# Autodesk Inventor assembly: In-Robot Assembly Full
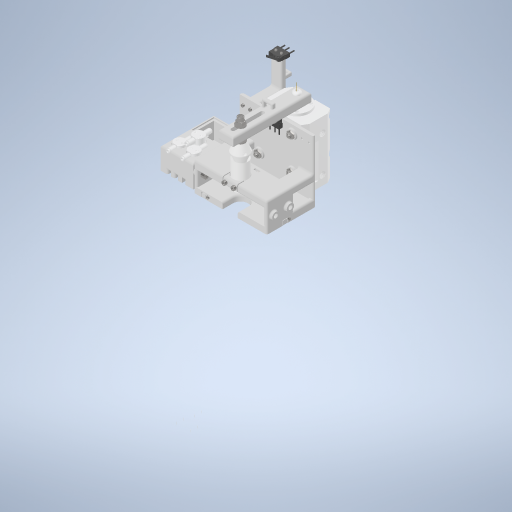
[picture p0: Inventor's stored thumbnail of the model, 512x512]
Saved by Autodesk Inventor 2024.1 (Build 281209000, 209)
## iProperties
Created: 2025-03-13
Part Number: In-Robot Assembly Full
Document SubType Name: Assembly
Designer: pab2
Author: pab2
## Documents named in this file (29)
- C:\Users\pab2\Documents\GitHub\AFL-hardware-devel\CAD-NewOrgScheme\AFL-101-(LoaderV2)\In-Robot Assembly Full.iam
- C:\Users\pab2\Documents\GitHub\AFL-hardware-devel\CAD-NewOrgScheme\AFL-101-(LoaderV2)\002-(CatchCarrierAssy)\AFL-101-002-01-0E CatchlessCatchHolder-Braced-For1inCatch-Sidebar-Lowered.ipt
- C:\Users\pab2\Documents\GitHub\AFL-hardware-devel\CAD-NewOrgScheme\AFL-101-(LoaderV2)\002-(CatchCarrierAssy)\AFL-101-002-01-4E RetainerNut.ipt
- C:\Users\pab2\Documents\GitHub\AFL-hardware-devel\CAD-NewOrgScheme\AFL-101-(LoaderV2)\002-(CatchCarrierAssy)\AFL-101-002-01-1A full-up microswitch arm.ipt
- C:\Users\pab2\Documents\GitHub\AFL-hardware-devel\CAD-NewOrgScheme\AFL-101-(LoaderV2)\002-(CatchCarrierAssy)\AFL-101-002-01-2B Elevator arm r2.ipt
- C:\Users\pab2\Documents\GitHub\AFL-hardware-devel\CAD-NewOrgScheme\AFL-101-(LoaderV2)\002-(CatchCarrierAssy)\AFL-101-002-01-3B CatchHolderNut.ipt
- C:\Users\pab2\Documents\GitHub\AFL-hardware-devel\CAD-NewOrgScheme\AFL-101-(LoaderV2)\001-(CatchAssy)\AFL-101-001-02-0C catch vertical seal-tighttol-thread - SANS.ipt
- C:\Users\pab2\Documents\GitHub\AFL-hardware-devel\CAD-NewOrgScheme\AFL-101-(LoaderV2)\001-(CatchAssy)\AFL-101-001-02-1C piston badflowchannel-1-16in-thread - neutron - 65flowchan.ipt
- C:\Users\pab2\Documents\GitHub\AFL-hardware-devel\CAD-NewOrgScheme\AFL-101-(LoaderV2)\003-(ValveBox)\AFL-101-003-01-0C Valve Holder-3valve-withwirebox-fortappedholes.ipt
- C:\Users\pab2\Downloads\50185A34_Air-Powered Hold-Down Fixture Clamp\50185A34_Air-Powered Hold-Down Fixture Clamp.ipt
- C:\Users\pab2\Downloads\5001T38_Miniature Solenoid On-Off Valve\5001T38_Miniature Solenoid On-Off Valve.ipt
- C:\Users\pab2\Downloads\8085T18_Subminiature Wet-Location Snap-Acting Switch\8085T18_Subminiature Wet-Location Snap-Acting Switch.ipt
- C:\Users\pab2\Documents\Inventor\Content Center Files\R2024\en-US\ANSI B18.2.2(09)\ANSI B18.2.2 - 1_4 - 20(2).ipt
- C:\Users\pab2\Documents\Inventor\Content Center Files\R2024\en-US\ANSI B18.3(05)\ANSI B18.3 - 1_4-20 UNC - 1.75(31).ipt
- C:\Users\pab2\Documents\Inventor\Content Center Files\R2024\en-US\ANSI B18.3(05)\ANSI B18.3 - 1_4-20 UNC - 0.25(31).ipt
- C:\Users\pab2\Documents\Inventor\Content Center Files\R2024\en-US\ANSI B18.3(05)\ANSI B18.3 - 8-32 UNC - 1.75(31).ipt
- C:\Users\pab2\Documents\Inventor\Content Center Files\R2024\en-US\ANSI B18.2.2(06)\ANSI B18.2.2 - 8 - 32(06).ipt
- C:\Users\pab2\Documents\Inventor\Content Center Files\R2024\en-US\ANSI B18.3(05)\ANSI B18.3 - 4-40 UNC - 0.25(31).ipt
- C:\Users\pab2\Documents\Inventor\Content Center Files\R2024\en-US\ANSI B18.3(05)\ANSI B18.3 - 2-56 UNC - 0.15625(31).ipt
- C:\Users\pab2\Documents\Inventor\Content Center Files\R2024\en-US\ANSI B18.3(05)\ANSI B18.3 - 4-40 UNC - 0.5(31).ipt
- C:\Users\pab2\Downloads\5779K241_Push-to-Connect Tube Fitting for Air\5779K241_Push-to-Connect Tube Fitting for Air.ipt
- C:\Users\pab2\Documents\Inventor\Content Center Files\R2024\en-US\ASTM F436(1)\ASTM F436 - 1_4(1).ipt
- C:\Users\pab2\Documents\Inventor\Content Center Files\R2024\en-US\ANSI B18.3(05)\ANSI B18.3 - 1_4-20 UNC - 1.5(31).ipt
- C:\Users\pab2\Documents\GitHub\AFL-hardware-devel\CAD-NewOrgScheme\AFL-101-(LoaderV2)\In-Robot Assembly Full\AIP\FEA\f06gvksv4.fins
- C:\Users\pab2\Documents\GitHub\AFL-hardware-devel\CAD-NewOrgScheme\AFL-101-(LoaderV2)\In-Robot Assembly Full\AIP\FEA\f06gvksw0.fsat
- C:\Users\pab2\Documents\GitHub\AFL-hardware-devel\CAD-NewOrgScheme\AFL-101-(LoaderV2)\In-Robot Assembly Full\AIP\FEA\f06gvksw0.ftes
- C:\Users\pab2\Documents\GitHub\AFL-hardware-devel\CAD-NewOrgScheme\AFL-101-(LoaderV2)\In-Robot Assembly Full\AIP\FEA\f06gvksw0.fwiz
- C:\Users\pab2\Documents\GitHub\AFL-hardware-devel\CAD-NewOrgScheme\AFL-101-(LoaderV2)\In-Robot Assembly Full\AIP\FEA\f06gvkta8.fmsh
- C:\Users\pab2\Documents\GitHub\AFL-hardware-devel\CAD-NewOrgScheme\AFL-101-(LoaderV2)\In-Robot Assembly Full\AIP\FEA\f06gvkta9.fres
## Components (49 placed, 22 different names)
1. AFL-101-002-01-0E CatchlessCatchHolder-Braced-For1inCatch-Sidebar-Lowered:1 — Mate:1, Mate:2, Mate:3, Mate:4, Mate:5, Mate:6, Mate:10, Flush:1, Mate:11, Flush:2, Mate:12, Mate:13, Mate:14, Mate:15, Mate:16, Mate:17, Mate:27, Mate:28, Mate:29, Insert:1, Insert:2, Insert:3, Insert:4, Insert:9, Insert:10, Insert:11, Insert:14, Insert:15, Insert:16, Insert:17, Insert:22, Insert:23
2. AFL-101-002-01-4E RetainerNut:1 — Mate:11, Flush:2
3. AFL-101-002-01-4E RetainerNut:2 — Mate:10, Flush:1
4. AFL-101-002-01-1A full-up microswitch arm:1 — Mate:12, Mate:13, Mate:14, Mate:24, Mate:25, Mate:26
5. AFL-101-002-01-2B Elevator arm r2:1 — Mate:18, Angle:1, Mate:42, Mate:44
6. AFL-101-002-01-3B CatchHolderNut:1 — Mate:7, Mate:8, Mate:9, Insert:12, Insert:13
7. AFL-101-001-02-0C catch vertical seal-tighttol-thread - SANS:1 — Mate:4, Mate:5, Mate:6, Mate:7, Mate:8, Mate:9, Mate:19
8. AFL-101-001-02-1C piston badflowchannel-1-16in-thread - neutron - 65flowchan:1 — Mate:19, Insert:24, Mate:43, Mate:44
9. AFL-101-003-01-0C Valve Holder-3valve-withwirebox-fortappedholes:1 — Mate:1, Mate:2, Mate:3, Mate:21, Mate:22, Mate:23
10. 50185A34_Air-Powered Hold-Down Fixture Clamp:1 — Mate:15, Mate:16, Mate:17, Mate:18, Angle:1, Insert:5, Insert:6, Insert:7, Insert:8
11. 5001T38_Miniature Solenoid On-Off Valve:1 — Mate:22, Mate:34, Mate:35, Mate:40, Mate:41
12. 5001T38_Miniature Solenoid On-Off Valve:2 — Mate:21, Mate:32, Mate:33, Mate:36, Mate:37
13. 5001T38_Miniature Solenoid On-Off Valve:3 — Mate:23, Mate:30, Mate:31, Mate:38, Mate:39
14. 8085T18_Subminiature Wet-Location Snap-Acting Switch:1 — Mate:27, Mate:28, Mate:29, Insert:20, Insert:21
15. 8085T18_Subminiature Wet-Location Snap-Acting Switch:2 — Mate:24, Mate:25, Mate:26, Insert:18, Insert:19
16. Hex Nut - Inch 1/4 - 20:1 — Insert:1
17. Hex Nut - Inch 1/4 - 20:2 — Insert:2
18. Hex Nut - Inch 1/4 - 20:3 — Insert:3
19. Hex Nut - Inch 1/4 - 20:4 — Insert:4
20. Hexagon Socket Head Cap Screw - Inch 1/4 - 20 UNC - 1 3/4:1 — Insert:5
21. Hexagon Socket Head Cap Screw - Inch 1/4 - 20 UNC - 1 3/4:2 — Insert:6
22. Hexagon Socket Head Cap Screw - Inch 1/4 - 20 UNC - 1 3/4:3 — Insert:7
23. Hexagon Socket Head Cap Screw - Inch 1/4 - 20 UNC - 1 3/4:4 — Insert:8
24. Hexagon Socket Head Cap Screw - Inch 1/4 - 20 UNC - 1/4:1 — Insert:9
25. Hexagon Socket Head Cap Screw - Inch 1/4 - 20 UNC - 1/4:2 — Insert:10
26. Hexagon Socket Head Cap Screw - Inch 1/4 - 20 UNC - 1/4:3 — Insert:11
27. Hexagon Socket Head Cap Screw - Inch No. 8 - 32 UNC - 1 3/4:1 — Insert:12
28. Hexagon Socket Head Cap Screw - Inch No. 8 - 32 UNC - 1 3/4:2 — Insert:13
29. Hex Machine Screw Nut - Inch 8 - 32:1 — Insert:14
30. Hex Machine Screw Nut - Inch 8 - 32:2 — Insert:15
31. Hexagon Socket Head Cap Screw - Inch No. 4 - 40 UNC - 1/4:2 — Insert:16
32. Hexagon Socket Head Cap Screw - Inch No. 4 - 40 UNC - 1/4:1 — Insert:17
33. Hexagon Socket Head Cap Screw - Inch No. 2 - 56 UNC - 5/32:1 — Insert:18
34. Hexagon Socket Head Cap Screw - Inch No. 2 - 56 UNC - 5/32:2 — Insert:19
35. Hexagon Socket Head Cap Screw - Inch No. 2 - 56 UNC - 5/32:3 — Insert:20
36. Hexagon Socket Head Cap Screw - Inch No. 2 - 56 UNC - 5/32:4 — Insert:21
37. Hexagon Socket Head Cap Screw - Inch No. 4 - 40 UNC - 1/2:2 — Insert:22
38. Hexagon Socket Head Cap Screw - Inch No. 4 - 40 UNC - 1/2:1 — Insert:23
39. 5779K241_Push-to-Connect Tube Fitting for Air:1 — Mate:32, Mate:33
40. 5779K241_Push-to-Connect Tube Fitting for Air:2 — Mate:36, Mate:37
41. 5779K241_Push-to-Connect Tube Fitting for Air:3 — Mate:34, Mate:35
42. 5779K241_Push-to-Connect Tube Fitting for Air:4 — Mate:30, Mate:31
43. 5779K241_Push-to-Connect Tube Fitting for Air:5 — Mate:38, Mate:39
44. 5779K241_Push-to-Connect Tube Fitting for Air:6 — Mate:40, Mate:41
45. Circular Washer (Inch) 1/4:1 — Insert:24, Insert:25
46. Hex Nut - Inch 1/4 - 20:5 — Insert:25
47. Circular Washer (Inch) 1/4:2 — Mate:42, Mate:43, Insert:26
48. Hex Nut - Inch 1/4 - 20:6 — Insert:26, Insert:27
49. Hexagon Socket Head Cap Screw - Inch 1/4 - 20 UNC - 1 1/2:1 — Insert:27
## Relationships (73: Mate 43, Insert 27, Flush 2, Angle 1)
- Mate:1: AFL-101-002-01-0E CatchlessCatchHolder-Braced-For1inCatch-Sidebar-Lowered:1 ↔ AFL-101-003-01-0C Valve Holder-3valve-withwirebox-fortappedholes:1
- Mate:2: AFL-101-002-01-0E CatchlessCatchHolder-Braced-For1inCatch-Sidebar-Lowered:1 ↔ AFL-101-003-01-0C Valve Holder-3valve-withwirebox-fortappedholes:1
- Mate:3: AFL-101-002-01-0E CatchlessCatchHolder-Braced-For1inCatch-Sidebar-Lowered:1 ↔ AFL-101-003-01-0C Valve Holder-3valve-withwirebox-fortappedholes:1
- Mate:4: AFL-101-002-01-0E CatchlessCatchHolder-Braced-For1inCatch-Sidebar-Lowered:1 ↔ AFL-101-001-02-0C catch vertical seal-tighttol-thread - SANS:1
- Mate:5: AFL-101-002-01-0E CatchlessCatchHolder-Braced-For1inCatch-Sidebar-Lowered:1 ↔ AFL-101-001-02-0C catch vertical seal-tighttol-thread - SANS:1
- Mate:6: AFL-101-002-01-0E CatchlessCatchHolder-Braced-For1inCatch-Sidebar-Lowered:1 ↔ AFL-101-001-02-0C catch vertical seal-tighttol-thread - SANS:1
- Mate:7: AFL-101-002-01-3B CatchHolderNut:1 ↔ AFL-101-001-02-0C catch vertical seal-tighttol-thread - SANS:1
- Mate:8: AFL-101-002-01-3B CatchHolderNut:1 ↔ AFL-101-001-02-0C catch vertical seal-tighttol-thread - SANS:1
- Mate:9: AFL-101-002-01-3B CatchHolderNut:1 ↔ AFL-101-001-02-0C catch vertical seal-tighttol-thread - SANS:1
- Mate:10: AFL-101-002-01-0E CatchlessCatchHolder-Braced-For1inCatch-Sidebar-Lowered:1 ↔ AFL-101-002-01-4E RetainerNut:2
- Flush:1: AFL-101-002-01-0E CatchlessCatchHolder-Braced-For1inCatch-Sidebar-Lowered:1 ↔ AFL-101-002-01-4E RetainerNut:2
- Mate:11: AFL-101-002-01-0E CatchlessCatchHolder-Braced-For1inCatch-Sidebar-Lowered:1 ↔ AFL-101-002-01-4E RetainerNut:1
- Flush:2: AFL-101-002-01-0E CatchlessCatchHolder-Braced-For1inCatch-Sidebar-Lowered:1 ↔ AFL-101-002-01-4E RetainerNut:1
- Mate:12: AFL-101-002-01-0E CatchlessCatchHolder-Braced-For1inCatch-Sidebar-Lowered:1 ↔ AFL-101-002-01-1A full-up microswitch arm:1
- Mate:13: AFL-101-002-01-0E CatchlessCatchHolder-Braced-For1inCatch-Sidebar-Lowered:1 ↔ AFL-101-002-01-1A full-up microswitch arm:1
- Mate:14: AFL-101-002-01-0E CatchlessCatchHolder-Braced-For1inCatch-Sidebar-Lowered:1 ↔ AFL-101-002-01-1A full-up microswitch arm:1
- Mate:15: AFL-101-002-01-0E CatchlessCatchHolder-Braced-For1inCatch-Sidebar-Lowered:1 ↔ 50185A34_Air-Powered Hold-Down Fixture Clamp:1
- Mate:16: AFL-101-002-01-0E CatchlessCatchHolder-Braced-For1inCatch-Sidebar-Lowered:1 ↔ 50185A34_Air-Powered Hold-Down Fixture Clamp:1
- Mate:17: AFL-101-002-01-0E CatchlessCatchHolder-Braced-For1inCatch-Sidebar-Lowered:1 ↔ 50185A34_Air-Powered Hold-Down Fixture Clamp:1
- Mate:18: AFL-101-002-01-2B Elevator arm r2:1 ↔ 50185A34_Air-Powered Hold-Down Fixture Clamp:1
- Angle:1 (90 deg): AFL-101-002-01-2B Elevator arm r2:1 ↔ 50185A34_Air-Powered Hold-Down Fixture Clamp:1
- Mate:19: AFL-101-001-02-0C catch vertical seal-tighttol-thread - SANS:1 ↔ AFL-101-001-02-1C piston badflowchannel-1-16in-thread - neutron - 65flowchan:1
- Mate:21: AFL-101-003-01-0C Valve Holder-3valve-withwirebox-fortappedholes:1 ↔ 5001T38_Miniature Solenoid On-Off Valve:2
- Mate:22: AFL-101-003-01-0C Valve Holder-3valve-withwirebox-fortappedholes:1 ↔ 5001T38_Miniature Solenoid On-Off Valve:1
- Mate:23: AFL-101-003-01-0C Valve Holder-3valve-withwirebox-fortappedholes:1 ↔ 5001T38_Miniature Solenoid On-Off Valve:3
- Mate:24: AFL-101-002-01-1A full-up microswitch arm:1 ↔ 8085T18_Subminiature Wet-Location Snap-Acting Switch:2
- Mate:25: AFL-101-002-01-1A full-up microswitch arm:1 ↔ 8085T18_Subminiature Wet-Location Snap-Acting Switch:2
- Mate:26: AFL-101-002-01-1A full-up microswitch arm:1 ↔ 8085T18_Subminiature Wet-Location Snap-Acting Switch:2
- Mate:27: AFL-101-002-01-0E CatchlessCatchHolder-Braced-For1inCatch-Sidebar-Lowered:1 ↔ 8085T18_Subminiature Wet-Location Snap-Acting Switch:1
- Mate:28: AFL-101-002-01-0E CatchlessCatchHolder-Braced-For1inCatch-Sidebar-Lowered:1 ↔ 8085T18_Subminiature Wet-Location Snap-Acting Switch:1
- Mate:29: AFL-101-002-01-0E CatchlessCatchHolder-Braced-For1inCatch-Sidebar-Lowered:1 ↔ 8085T18_Subminiature Wet-Location Snap-Acting Switch:1
- Insert:1: AFL-101-002-01-0E CatchlessCatchHolder-Braced-For1inCatch-Sidebar-Lowered:1 ↔ Hex Nut - Inch 1/4 - 20:1
- Insert:2: AFL-101-002-01-0E CatchlessCatchHolder-Braced-For1inCatch-Sidebar-Lowered:1 ↔ Hex Nut - Inch 1/4 - 20:2
- Insert:3: AFL-101-002-01-0E CatchlessCatchHolder-Braced-For1inCatch-Sidebar-Lowered:1 ↔ Hex Nut - Inch 1/4 - 20:3
- Insert:4: AFL-101-002-01-0E CatchlessCatchHolder-Braced-For1inCatch-Sidebar-Lowered:1 ↔ Hex Nut - Inch 1/4 - 20:4
- Insert:5: 50185A34_Air-Powered Hold-Down Fixture Clamp:1 ↔ Hexagon Socket Head Cap Screw - Inch 1/4 - 20 UNC - 1 3/4:1
- Insert:6: 50185A34_Air-Powered Hold-Down Fixture Clamp:1 ↔ Hexagon Socket Head Cap Screw - Inch 1/4 - 20 UNC - 1 3/4:2
- Insert:7: 50185A34_Air-Powered Hold-Down Fixture Clamp:1 ↔ Hexagon Socket Head Cap Screw - Inch 1/4 - 20 UNC - 1 3/4:3
- Insert:8: 50185A34_Air-Powered Hold-Down Fixture Clamp:1 ↔ Hexagon Socket Head Cap Screw - Inch 1/4 - 20 UNC - 1 3/4:4
- Insert:9: AFL-101-002-01-0E CatchlessCatchHolder-Braced-For1inCatch-Sidebar-Lowered:1 ↔ Hexagon Socket Head Cap Screw - Inch 1/4 - 20 UNC - 1/4:1
- Insert:10: AFL-101-002-01-0E CatchlessCatchHolder-Braced-For1inCatch-Sidebar-Lowered:1 ↔ Hexagon Socket Head Cap Screw - Inch 1/4 - 20 UNC - 1/4:2
- Insert:11: AFL-101-002-01-0E CatchlessCatchHolder-Braced-For1inCatch-Sidebar-Lowered:1 ↔ Hexagon Socket Head Cap Screw - Inch 1/4 - 20 UNC - 1/4:3
- Insert:12: AFL-101-002-01-3B CatchHolderNut:1 ↔ Hexagon Socket Head Cap Screw - Inch No. 8 - 32 UNC - 1 3/4:1
- Insert:13: AFL-101-002-01-3B CatchHolderNut:1 ↔ Hexagon Socket Head Cap Screw - Inch No. 8 - 32 UNC - 1 3/4:2
- Insert:14: AFL-101-002-01-0E CatchlessCatchHolder-Braced-For1inCatch-Sidebar-Lowered:1 ↔ Hex Machine Screw Nut - Inch 8 - 32:1
- Insert:15: AFL-101-002-01-0E CatchlessCatchHolder-Braced-For1inCatch-Sidebar-Lowered:1 ↔ Hex Machine Screw Nut - Inch 8 - 32:2
- Insert:16: AFL-101-002-01-0E CatchlessCatchHolder-Braced-For1inCatch-Sidebar-Lowered:1 ↔ Hexagon Socket Head Cap Screw - Inch No. 4 - 40 UNC - 1/4:2
- Insert:17: AFL-101-002-01-0E CatchlessCatchHolder-Braced-For1inCatch-Sidebar-Lowered:1 ↔ Hexagon Socket Head Cap Screw - Inch No. 4 - 40 UNC - 1/4:1
- Insert:18: 8085T18_Subminiature Wet-Location Snap-Acting Switch:2 ↔ Hexagon Socket Head Cap Screw - Inch No. 2 - 56 UNC - 5/32:1
- Insert:19: 8085T18_Subminiature Wet-Location Snap-Acting Switch:2 ↔ Hexagon Socket Head Cap Screw - Inch No. 2 - 56 UNC - 5/32:2
- Insert:20: 8085T18_Subminiature Wet-Location Snap-Acting Switch:1 ↔ Hexagon Socket Head Cap Screw - Inch No. 2 - 56 UNC - 5/32:3
- Insert:21: 8085T18_Subminiature Wet-Location Snap-Acting Switch:1 ↔ Hexagon Socket Head Cap Screw - Inch No. 2 - 56 UNC - 5/32:4
- Insert:22: AFL-101-002-01-0E CatchlessCatchHolder-Braced-For1inCatch-Sidebar-Lowered:1 ↔ Hexagon Socket Head Cap Screw - Inch No. 4 - 40 UNC - 1/2:2
- Insert:23: AFL-101-002-01-0E CatchlessCatchHolder-Braced-For1inCatch-Sidebar-Lowered:1 ↔ Hexagon Socket Head Cap Screw - Inch No. 4 - 40 UNC - 1/2:1
- Mate:30: 5001T38_Miniature Solenoid On-Off Valve:3 ↔ 5779K241_Push-to-Connect Tube Fitting for Air:4
- Mate:31: 5001T38_Miniature Solenoid On-Off Valve:3 ↔ 5779K241_Push-to-Connect Tube Fitting for Air:4
- Mate:32: 5001T38_Miniature Solenoid On-Off Valve:2 ↔ 5779K241_Push-to-Connect Tube Fitting for Air:1
- Mate:33: 5001T38_Miniature Solenoid On-Off Valve:2 ↔ 5779K241_Push-to-Connect Tube Fitting for Air:1
- Mate:34: 5001T38_Miniature Solenoid On-Off Valve:1 ↔ 5779K241_Push-to-Connect Tube Fitting for Air:3
- Mate:35: 5001T38_Miniature Solenoid On-Off Valve:1 ↔ 5779K241_Push-to-Connect Tube Fitting for Air:3
- Mate:36: 5001T38_Miniature Solenoid On-Off Valve:2 ↔ 5779K241_Push-to-Connect Tube Fitting for Air:2
- Mate:37: 5001T38_Miniature Solenoid On-Off Valve:2 ↔ 5779K241_Push-to-Connect Tube Fitting for Air:2
- Mate:38: 5001T38_Miniature Solenoid On-Off Valve:3 ↔ 5779K241_Push-to-Connect Tube Fitting for Air:5
- Mate:39: 5001T38_Miniature Solenoid On-Off Valve:3 ↔ 5779K241_Push-to-Connect Tube Fitting for Air:5
- Mate:40: 5001T38_Miniature Solenoid On-Off Valve:1 ↔ 5779K241_Push-to-Connect Tube Fitting for Air:6
- Mate:41: 5001T38_Miniature Solenoid On-Off Valve:1 ↔ 5779K241_Push-to-Connect Tube Fitting for Air:6
- Insert:24: AFL-101-001-02-1C piston badflowchannel-1-16in-thread - neutron - 65flowchan:1 ↔ Circular Washer (Inch) 1/4:1
- Insert:25: Circular Washer (Inch) 1/4:1 ↔ Hex Nut - Inch 1/4 - 20:5
- Mate:42: AFL-101-002-01-2B Elevator arm r2:1 ↔ Circular Washer (Inch) 1/4:2
- Mate:43: AFL-101-001-02-1C piston badflowchannel-1-16in-thread - neutron - 65flowchan:1 ↔ Circular Washer (Inch) 1/4:2
- Insert:26: Circular Washer (Inch) 1/4:2 ↔ Hex Nut - Inch 1/4 - 20:6
- Insert:27: Hex Nut - Inch 1/4 - 20:6 ↔ Hexagon Socket Head Cap Screw - Inch 1/4 - 20 UNC - 1 1/2:1
- Mate:44 (7.62 mm): AFL-101-002-01-2B Elevator arm r2:1 ↔ AFL-101-001-02-1C piston badflowchannel-1-16in-thread - neutron - 65flowchan:1
## Named parameters: sa_0 = 13344.7
note: some values were not read from the file. Shown as the stored number, unit unknown: "sa_0".
